# Autodesk Inventor assembly: PMax8
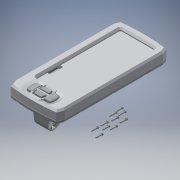
[picture p0: Inventor's stored thumbnail of the model, 180x180]
Saved by Autodesk Inventor 2018 (Build 220112000, 112)
## iProperties
Created: 2019-05-29
Part Number: PMax8
Document SubType Name: Assembly
Designer: Ash
Author: Ash
## Documents named in this file (8)
- C:\Autodesk\Skills 2019 Nationals\Competition\PMDay2\PMax8.iam
- C:\Autodesk\Skills 2019 Nationals\Competition\PMDay2\#2-KEYPAD.ipt
- C:\Autodesk\Skills 2019 Nationals\Competition\PMDay1\Front_Cover3.ipt
- C:\Autodesk\Skills 2019 Nationals\Competition\PMDay1\Display_Plate3.ipt
- C:\Autodesk\Skills 2019 Nationals\Competition\PMDay2\#4-GASKET(PMAX8).ipt
- C:\Autodesk\Skills 2019 Nationals\Competition\PMDay2\#5-BACK_COVER(PMAX8).ipt
- C:\Autodesk\Skills 2019 Nationals\Competition\PMDay2\ADDITIONAL_BUTTON.ipt
- C:\Autodesk\Skills 2019 Nationals\Competition\PMDay2\#6-SCREW.ipt
## Components (16 placed, 7 different names)
1. #2-KEYPAD:1 — Mate:6, Mate:7, Mate:8, Mate:9, Mate:11
2. Display_Plate3:1 — Mate:7, Mate:10, Mate:11
3. Front_Cover3:1 — Mate:6, Mate:8, Mate:9, Mate:10, Mate:15, Mate:16, Mate:17, Mate:18, Flush:1
4. #4-GASKET(PMAX8):1 — Mate:12, Mate:13, Mate:14, Mate:19
5. #5-BACK_COVER(PMAX8):1 — Mate:12, Mate:13, Mate:14, Mate:15, Mate:16, Mate:17
6. ADDITIONAL_BUTTON:1 — Mate:18, Mate:19, Flush:1
7. #6-SCREW:1
8. #6-SCREW:2
9. #6-SCREW:3
10. #6-SCREW:4
11. #6-SCREW:5
12. #6-SCREW:6
13. #6-SCREW:7
14. #6-SCREW:8
15. #6-SCREW:9
16. #6-SCREW:10
## Relationships (15: Mate 14, Flush 1)
- Mate:6 (6.35 mm): #2-KEYPAD:1 ↔ Front_Cover3:1
- Mate:7: #2-KEYPAD:1 ↔ Display_Plate3:1
- Mate:8: #2-KEYPAD:1 ↔ Front_Cover3:1
- Mate:9 (46.7868 mm): #2-KEYPAD:1 ↔ Front_Cover3:1
- Mate:10: Display_Plate3:1 ↔ Front_Cover3:1
- Mate:11: #2-KEYPAD:1 ↔ Display_Plate3:1
- Mate:12: #4-GASKET(PMAX8):1 ↔ #5-BACK_COVER(PMAX8):1
- Mate:13: #4-GASKET(PMAX8):1 ↔ #5-BACK_COVER(PMAX8):1
- Mate:14: #4-GASKET(PMAX8):1 ↔ #5-BACK_COVER(PMAX8):1
- Mate:15: Front_Cover3:1 ↔ #5-BACK_COVER(PMAX8):1
- Mate:16: Front_Cover3:1 ↔ #5-BACK_COVER(PMAX8):1
- Mate:17: Front_Cover3:1 ↔ #5-BACK_COVER(PMAX8):1
- Mate:18 (-10.16 mm): Front_Cover3:1 ↔ ADDITIONAL_BUTTON:1
- Mate:19 (6.35 mm): #4-GASKET(PMAX8):1 ↔ ADDITIONAL_BUTTON:1
- Flush:1: Front_Cover3:1 ↔ ADDITIONAL_BUTTON:1
